# Autodesk Inventor assembly: Cart
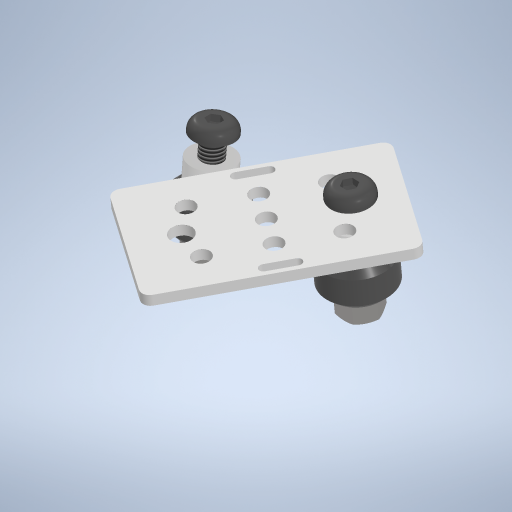
[picture p0: Inventor's stored thumbnail of the model, 512x512]
Saved by Autodesk Inventor 2024 (Build 280153000, 153)
## iProperties
Created: 2024-12-08
Part Number: Cart
Document SubType Name: Assembly
Designer: Nada
Author: Nada
## Documents named in this file (3)
- C:\Users\Adham\Desktop\Modelling Project\Repo\Online-Parameter-Estimation\CAD\Cart\Cart.iam
- C:\Users\Adham\Desktop\Modelling Project\Repo\Online-Parameter-Estimation\CAD\Cart\Cart.ipt
- C:\Users\Adham\Desktop\Modelling Project\Repo\Online-Parameter-Estimation\CAD\Cart\Delrin Mini V-Wheel.iam
## Components (3 placed, 2 different names)
1. Cart:1 — Mate:1
2. Delrin Mini V-Wheel:1 [sub-assembly] — Mate:1
3. Delrin Mini V-Wheel:2 [sub-assembly]
## Relationships (1: Mate 1)
- Mate:1: Cart:1 ↔ Delrin Mini V-Wheel:1
